# Autodesk Inventor assembly: table
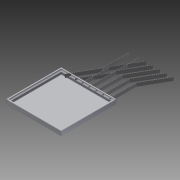
[picture p0: Inventor's stored thumbnail of the model, 180x180]
Saved by Autodesk Inventor 2013 (Build 170138000, 138)
## iProperties
Created: 2012-10-20
Part Number: table
Document SubType Name: Weldment
Designer: Istvan
Weld Material: Welded Aluminum-6061
Mass: 18318.1 g
Surface Area: 68009.8 cm^2
Volume: 8886.11 cm^3
Density: 2.06143 g/cm^3
Author: Istvan
## Documents named in this file (7)
- C:\Users\istvan.burbank\Documents\GitHub\Crown-Fire\CAD\Frame\Table\table.iam
- C:\Users\istvan.burbank\Documents\GitHub\Crown-Fire\CAD\Frame\Table\tableBottom.ipt
- C:\Users\istvan.burbank\Documents\GitHub\Crown-Fire\CAD\Frame\Table\tableSide.ipt
- C:\Users\istvan.burbank\Documents\GitHub\Crown-Fire\CAD\Templates\squareTube1.5x2.ipt
- C:\Users\istvan.burbank\Documents\GitHub\Crown-Fire\CAD\Frame\Table\slatHolder.ipt
- C:\Users\istvan.burbank\Documents\GitHub\Crown-Fire\CAD\Frame\Table\slatHolderShort.ipt
- C:\Users\istvan.burbank\Documents\GitHub\Crown-Fire\CAD\Frame\Table\slats.ipt
## Components (16 placed, 5 different names)
1. tableBottom:1 — Mate:38, Mate:39, Mate:40, Mate:41, Mate:48, Mate:49, Mate:50, Mate:51
2. tableSide:1 — Mate:40, Mate:44, Mate:45, Mate:46, Mate:47, Mate:49
3. tableSide:2 — Mate:41, Mate:46, Mate:47
4. tableSide:3 — Mate:39, Mate:42, Mate:43, Mate:44, Mate:45, Mate:48, Mate:57
5. tableSide:4 — Mate:38, Mate:42, Mate:43, Mate:56
6. slatHolder:2 — Flush:5, Mate:52, Mate:53, Flush:6, Flush:8, Mate:57
7. slatHolder:4 — Flush:3, Flush:4, Mate:54, Mate:55, Flush:7, Flush:9
8. slatHolderShort:6 — Mate:50, Flush:3, Mate:53, Mate:55, Flush:8, Flush:9, Mate:58, Mate:59, Mate:60, Mate:62, Mate:63
9. slatHolderShort:7 — Mate:51, Flush:4, Flush:5, Mate:52, Mate:54, Flush:6, Flush:7, Mate:56
10. slats:1 — Mate:58
11. slats:2 — Mate:59
12. slats:3 — Mate:63
13. slats:4 — Mate:60
14. slats:5 — Mate:62
15. slats:6
16. slats:7
## Relationships (32: Mate 25, Flush 7)
- Mate:38: tableBottom:1 ↔ tableSide:4
- Mate:39: tableBottom:1 ↔ tableSide:3
- Mate:40: tableBottom:1 ↔ tableSide:1
- Mate:41: tableBottom:1 ↔ tableSide:2
- Mate:42: tableSide:3 ↔ tableSide:4
- Mate:43: tableSide:3 ↔ tableSide:4
- Mate:44: tableSide:1 ↔ tableSide:3
- Mate:45: tableSide:1 ↔ tableSide:3
- Mate:46: tableSide:1 ↔ tableSide:2
- Mate:47: tableSide:1 ↔ tableSide:2
- Mate:48: tableBottom:1 ↔ tableSide:3
- Mate:49: tableBottom:1 ↔ tableSide:1
- Mate:50: tableBottom:1 ↔ slatHolderShort:6
- Mate:51: tableBottom:1 ↔ slatHolderShort:7
- Flush:3: slatHolder:4 ↔ slatHolderShort:6
- Flush:4: slatHolder:4 ↔ slatHolderShort:7
- Flush:5: slatHolder:2 ↔ slatHolderShort:7
- Mate:52: slatHolder:2 ↔ slatHolderShort:7
- Mate:53: slatHolder:2 ↔ slatHolderShort:6
- Mate:54: slatHolder:4 ↔ slatHolderShort:7
- Mate:55: slatHolder:4 ↔ slatHolderShort:6
- Flush:6: slatHolder:2 ↔ slatHolderShort:7
- Flush:7: slatHolder:4 ↔ slatHolderShort:7
- Flush:8: slatHolder:2 ↔ slatHolderShort:6
- Flush:9: slatHolder:4 ↔ slatHolderShort:6
- Mate:56: tableSide:4 ↔ slatHolderShort:7
- Mate:57: tableSide:3 ↔ slatHolder:2
- Mate:58: slatHolderShort:6 ↔ slats:1
- Mate:59: slatHolderShort:6 ↔ slats:2
- Mate:60: slatHolderShort:6 ↔ slats:4
- Mate:62: slatHolderShort:6 ↔ slats:5
- Mate:63: slatHolderShort:6 ↔ slats:3
